# Autodesk Inventor assembly: SideChestPanel
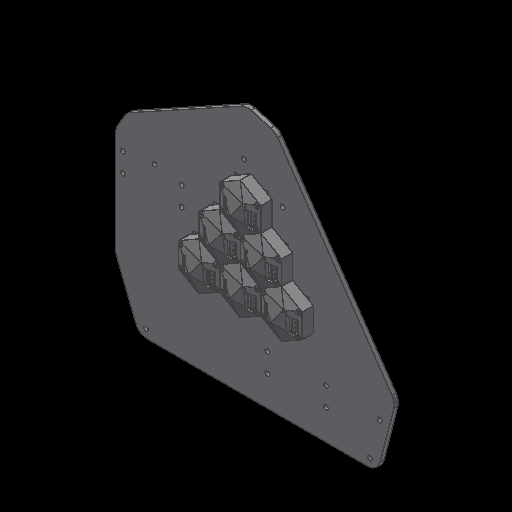
[picture p0: Inventor's stored thumbnail of the model, 512x512]
Saved by Autodesk Inventor 2025.2 (Build 292293000, 293)
## iProperties
Created: 2025-12-14
Part Number: SideChestPanel
Document SubType Name: Assembly
Designer: valer
Author: valer
## Documents named in this file (3)
- C:\Users\valer\Desktop\str1ker\cad\SideChestPanel.iam
- C:\Users\valer\Desktop\str1ker\cad\SideChestPanel.ipt
- C:\Users\valer\Desktop\str1ker\cad\ArmDriver.iam
## Components (7 placed, 2 different names)
1. SideChestPanel:1 — Flush:2, Flush:3, Flush:4, Mate:1, Mate:2, Mate:3, Mate:4, Mate:5, Mate:6, Mate:7, Mate:8, Mate:9, Mate:10, Mate:11, Mate:12, Mate:13, Mate:14, Mate:15, Mate:16, Mate:17
2. ArmDriver:1 [sub-assembly] — Mate:7, Mate:8, Mate:9
3. ArmDriver:2 [sub-assembly] — Mate:4, Mate:5, Mate:6
4. ArmDriver:3 [sub-assembly] — Mate:1, Mate:2, Mate:3, Angle:1
5. ArmDriver:4 [sub-assembly] — Mate:16, Mate:17, Angle:1
6. ArmDriver:5 [sub-assembly] — Mate:10, Mate:11, Mate:12
7. ArmDriver:6 [sub-assembly] — Mate:13, Mate:14, Mate:15
## Relationships (21: Mate 17, Flush 3, Angle 1)
- Flush:2: SideChestPanel:1
- Flush:3: SideChestPanel:1
- Flush:4: SideChestPanel:1
- Mate:1: SideChestPanel:1 ↔ ArmDriver:3
- Mate:2: SideChestPanel:1 ↔ ArmDriver:3
- Mate:3: SideChestPanel:1 ↔ ArmDriver:3
- Mate:4: SideChestPanel:1 ↔ ArmDriver:2
- Mate:5: SideChestPanel:1 ↔ ArmDriver:2
- Mate:6: SideChestPanel:1 ↔ ArmDriver:2
- Mate:7: SideChestPanel:1 ↔ ArmDriver:1
- Mate:8: SideChestPanel:1 ↔ ArmDriver:1
- Mate:9: SideChestPanel:1 ↔ ArmDriver:1
- Mate:10: SideChestPanel:1 ↔ ArmDriver:5
- Mate:11: SideChestPanel:1 ↔ ArmDriver:5
- Mate:12: SideChestPanel:1 ↔ ArmDriver:5
- Mate:13: SideChestPanel:1 ↔ ArmDriver:6
- Mate:14: SideChestPanel:1 ↔ ArmDriver:6
- Mate:15: SideChestPanel:1 ↔ ArmDriver:6
- Mate:16: SideChestPanel:1 ↔ ArmDriver:4
- Mate:17: SideChestPanel:1 ↔ ArmDriver:4
- Angle:1 (0 deg): ArmDriver:3 ↔ ArmDriver:4
